# Autodesk Inventor assembly: Wood_X_Frame
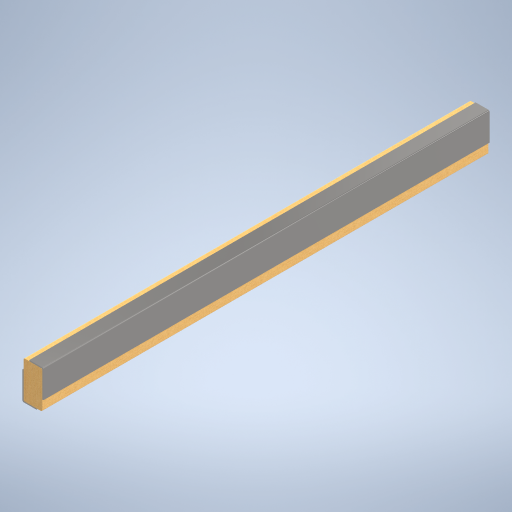
[picture p0: Inventor's stored thumbnail of the model, 512x512]
Saved by Autodesk Inventor 2023 (Build 270158000, 158)
## iProperties
Created: 2022-05-10
Part Number: Wood_X_Frame
Document SubType Name: Assembly
Designer: a laptop
Author: a laptop
## Documents named in this file (11)
- C:\Users\a laptop\Desktop\CNC_Project\Wood_X_Frame.iam
- C:\Users\a laptop\Desktop\CNC_Project\L_Channel.ipt
- C:\Users\a laptop\Desktop\CNC_Project\2x4_Wood.ipt
- C:\Users\a laptop\Desktop\CNC_Project\Wood_X_Frame\AIP\FEA\dytmg7jgg.fins
- C:\Users\a laptop\Desktop\CNC_Project\Wood_X_Frame\AIP\FEA\dytmg7jgg.fsat
- C:\Users\a laptop\Desktop\CNC_Project\Wood_X_Frame\AIP\FEA\dytmg7jhc.ftes
- C:\Users\a laptop\Desktop\CNC_Project\Wood_X_Frame\AIP\FEA\dytmg7jhc.fwiz
- C:\Users\a laptop\Desktop\CNC_Project\Wood_X_Frame\AIP\FEA\dytmg7jkw.fmsh
- C:\Users\a laptop\Desktop\CNC_Project\Wood_X_Frame\AIP\FEA\dytmg7jkx.fres
- C:\Users\a laptop\Desktop\CNC_Project\Wood_X_Frame\AIP\FEA\dytmg7jpc.fmsh
- C:\Users\a laptop\Desktop\CNC_Project\Wood_X_Frame\AIP\FEA\dytmg7jq8.fres
## Components (3 placed, 2 different names)
1. L_Channel:1
2. 2x4_Wood:1
3. L_Channel:2
## Relationships (6: Mate 4, Flush 2)
- [Mate]: L_Channel:1 ↔ 2x4_Wood:1
- [Mate]: L_Channel:1 ↔ 2x4_Wood:1
- [Flush]: L_Channel:1 ↔ 2x4_Wood:1
- [Flush]: 2x4_Wood:1 ↔ L_Channel:2
- [Mate]: 2x4_Wood:1 ↔ L_Channel:2
- [Mate]: 2x4_Wood:1 ↔ L_Channel:2
## Named parameters: sa_1 = 58800, sa_0 = 100000
note: some values were not read from the file. Shown as the stored number, unit unknown: "sa_1", "sa_0".
